# Autodesk Inventor assembly: Claw Assy
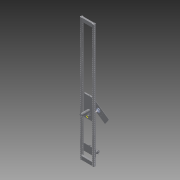
[picture p0: Inventor's stored thumbnail of the model, 180x180]
Saved by Autodesk Inventor 2015 (Build 190159000, 159)
## iProperties
Created: 2015-01-20
Part Number: Claw Assy
Document SubType Name: Assembly
Designer: chappelled
Author: chappelled
## Documents named in this file (8)
- \\lhssvr02\Homedirs\Robotics Club\CAD Model 2015\Claw Doug\Claw Assy.iam
- \\lhssvr02\Homedirs\Robotics Club\CAD Model 2015\Claw Doug\Frame.iam
- \\lhssvr02\Homedirs\Robotics Club\CAD Model 2015\Claw Doug\Motor Mount Assy.iam
- \\lhssvr02\Homedirs\Robotics Club\CAD Model 2015\Claw Doug\Spacer.ipt
- \\lhssvr02\Homedirs\Robotics Club\CAD Model 2015\Claw Doug\Claw Assy\Design Accelerator\Bolted Connection4.iam
- \\lhssvr02\Homedirs\Robotics Club\CAD Model 2015\Claw Doug\Traveler Assya.iam
- \\lhssvr02\Homedirs\Robotics Club\CAD Model 2015\Claw Doug\1x2x6.ipt
- \\lhssvr02\Homedirs\Robotics Club\CAD Model 2015\Claw Doug\Claw Plate Assy.iam
## Components (14 placed, 7 different names)
1. Frame:1 [sub-assembly] — Mate:1, Mate:2, Mate:3, Mate:4, Flush:2, Mate:8, Mate:10, Flush:4, Flush:5, Mate:12
2. Motor Mount Assy:1 [sub-assembly] — Mate:1, Mate:2, Mate:3, Mate:5, Mate:6, Mate:7
3. Traveler Assya:1 [sub-assembly] — Flush:1, Mate:8, Mate:13, Mate:14, Mate:17
4. 1x2x6:1 — Mate:10, Flush:3, Flush:4
5. 1x2x6:2 — Flush:5, Mate:12, Flush:6
6. Claw Plate Assy:1 [sub-assembly] — Mate:13, Mate:14, Mate:17
7. Spacer:1 — Mate:4, Mate:5
8. Spacer:2
9. Spacer:3
10. Spacer:4
11. Bolted Connection:1 [sub-assembly] — Mate:6, Mate:7
12. Bolted Connection:2 [sub-assembly]
13. Bolted Connection:3 [sub-assembly]
14. Bolted Connection:4 [sub-assembly]
## Component patterns: (4 elements, first: Spacer:1), (4 elements, first: Bolted Connection:1)
## Relationships (22: Mate 15, Flush 7)
- Mate:1 (6.35 mm): Frame:1 ↔ Motor Mount Assy:1
- Mate:2: Frame:1 ↔ Motor Mount Assy:1
- Mate:3: Frame:1 ↔ Motor Mount Assy:1
- Mate:4: Frame:1 ↔ Spacer:1
- Mate:5: Motor Mount Assy:1 ↔ Spacer:1
- Mate:6: Motor Mount Assy:1 ↔ Bolted Connection:1
- Mate:7: Motor Mount Assy:1 ↔ Bolted Connection:1
- Flush:1 (-76.2 mm): Traveler Assya:1
- Flush:2 (-104.775 mm): Frame:1
- Mate:8 (2.54 mm): Frame:1 ↔ Traveler Assya:1
- Mate:9
- Mate:10: Frame:1 ↔ 1x2x6:1
- Flush:3 (-98.425 mm): 1x2x6:1
- Mate:11
- Flush:4: Frame:1 ↔ 1x2x6:1
- Flush:5: Frame:1 ↔ 1x2x6:2
- Mate:12: Frame:1 ↔ 1x2x6:2
- Flush:6 (-98.425 mm): 1x2x6:2
- Flush:7
- Mate:13: Traveler Assya:1 ↔ Claw Plate Assy:1
- Mate:14: Traveler Assya:1 ↔ Claw Plate Assy:1
- Mate:17: Traveler Assya:1 ↔ Claw Plate Assy:1
